# Autodesk Inventor assembly: cabeça_superior
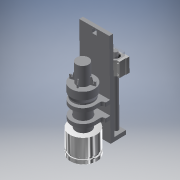
[picture p0: Inventor's stored thumbnail of the model, 180x180]
Saved by Autodesk Inventor 2018 (Build 220112000, 112)
## iProperties
Created: 2018-05-10
Part Number: cabeça_superior
Material: Genérico
Document SubType Name: Assembly
Designer: Georgines
Mass: 943.179 g
Surface Area: 3340.88 cm^2
Volume: 704.097 cm^3
Density: 1.33956 g/cm^3
Author: Georgines
## Documents named in this file (9)
- C:\Users\Georgines\Documents\EstacaoBGA\Peças 3D\cabeça_superior.iam
- C:\Users\Georgines\Documents\EstacaoBGA\Peças 3D\bocal_de_aquecimento.ipt
- C:\Users\Georgines\Documents\EstacaoBGA\Peças 3D\soprador_original.ipt
- C:\Users\Georgines\Documents\EstacaoBGA\Peças 3D\base_fixaxao_cabeca_supeior.ipt
- C:\Users\Georgines\Documents\EstacaoBGA\Peças 3D\carcaca_bocal_superior.ipt
- C:\Users\Georgines\Documents\EstacaoBGA\Peças 3D\SuporteGuiasCabeçasAquecimento.ipt
- C:\Users\Georgines\Documents\EstacaoBGA\Peças 3D\GuiaLinear_12x200mm.ipt
- C:\Users\Georgines\Documents\EstacaoBGA\Peças 3D\SCS12UU.iam
- C:\Users\Georgines\Documents\EstacaoBGA\Peças 3D\SuporteAquecedor.ipt
## Components (12 placed, 8 different names)
1. bocal_de_aquecimento:1 — Coincidência:16, Alinhamento:14, Coincidência:22
2. soprador_original:1 — Coincidência:15, Coincidência:16, Alinhamento:14, Coincidência:17
3. SuporteGuiasCabeçasAquecimento:1 — Coincidência:1, Coincidência:2, Alinhamento:13, Coincidência:19, Coincidência:20, Alinhamento:18, Alinhamento:19
4. SuporteGuiasCabeçasAquecimento:2 — Coincidência:3, Coincidência:4, Coincidência:11, Alinhamento:9, Alinhamento:20
5. GuiaLinear_12x200mm:1 — Coincidência:2, Coincidência:4, Coincidência:10, Alinhamento:19
6. GuiaLinear_12x200mm:2 — Coincidência:1, Coincidência:3, Coincidência:21, Alinhamento:18, Alinhamento:20
7. SCS12UU:1 [sub-assembly] — Coincidência:10, Coincidência:20, Alinhamento:16, Alinhamento:17
8. SCS12UU:4 [sub-assembly] — Coincidência:21, Alinhamento:16, Alinhamento:17
9. base_fixaxao_cabeca_supeior:1 — Coincidência:11, Alinhamento:9, Coincidência:12, Alinhamento:10, Coincidência:13, Alinhamento:11, Alinhamento:12, Alinhamento:13, Coincidência:18, Alinhamento:15, Coincidência:22
10. SuporteAquecedor:1 — Coincidência:12, Alinhamento:10, Alinhamento:12, Coincidência:14, Coincidência:15, Coincidência:17
11. SuporteAquecedor:2 — Coincidência:13, Alinhamento:11, Coincidência:14
12. carcaca_bocal_superior:1 — Coincidência:18, Coincidência:19, Alinhamento:15
## Relationships (29: Mate 17, Flush 12)
- Coincidência:1 [Mate]: SuporteGuiasCabeçasAquecimento:1 ↔ GuiaLinear_12x200mm:2
- Coincidência:2 [Mate]: SuporteGuiasCabeçasAquecimento:1 ↔ GuiaLinear_12x200mm:1
- Coincidência:3 [Mate]: SuporteGuiasCabeçasAquecimento:2 ↔ GuiaLinear_12x200mm:2
- Coincidência:4 [Mate]: SuporteGuiasCabeçasAquecimento:2 ↔ GuiaLinear_12x200mm:1
- Coincidência:10 [Mate]: GuiaLinear_12x200mm:1 ↔ SCS12UU:1
- Coincidência:11 [Mate]: SuporteGuiasCabeçasAquecimento:2 ↔ base_fixaxao_cabeca_supeior:1
- Alinhamento:9 [Flush]: SuporteGuiasCabeçasAquecimento:2 ↔ base_fixaxao_cabeca_supeior:1
- Coincidência:12 [Mate]: base_fixaxao_cabeca_supeior:1 ↔ SuporteAquecedor:1
- Alinhamento:10 [Flush]: base_fixaxao_cabeca_supeior:1 ↔ SuporteAquecedor:1
- Coincidência:13 [Mate]: base_fixaxao_cabeca_supeior:1 ↔ SuporteAquecedor:2
- Alinhamento:11 [Flush]: base_fixaxao_cabeca_supeior:1 ↔ SuporteAquecedor:2
- Alinhamento:12 [Flush] (142.072 mm): base_fixaxao_cabeca_supeior:1 ↔ SuporteAquecedor:1
- Coincidência:14 [Mate] (25.75 mm): SuporteAquecedor:1 ↔ SuporteAquecedor:2
- Alinhamento:13 [Flush]: SuporteGuiasCabeçasAquecimento:1 ↔ base_fixaxao_cabeca_supeior:1
- Coincidência:15 [Mate]: soprador_original:1 ↔ SuporteAquecedor:1
- Coincidência:16 [Mate]: bocal_de_aquecimento:1 ↔ soprador_original:1
- Alinhamento:14 [Flush] (2.5 mm): bocal_de_aquecimento:1 ↔ soprador_original:1
- Coincidência:17 [Mate] (5 mm): soprador_original:1 ↔ SuporteAquecedor:1
- Coincidência:18 [Mate]: base_fixaxao_cabeca_supeior:1 ↔ carcaca_bocal_superior:1
- Coincidência:19 [Mate]: SuporteGuiasCabeçasAquecimento:1 ↔ carcaca_bocal_superior:1
- Alinhamento:15 [Flush]: base_fixaxao_cabeca_supeior:1 ↔ carcaca_bocal_superior:1
- Coincidência:20 [Mate]: SuporteGuiasCabeçasAquecimento:1 ↔ SCS12UU:1
- Coincidência:21 [Mate]: GuiaLinear_12x200mm:2 ↔ SCS12UU:4
- Alinhamento:16 [Flush]: SCS12UU:1 ↔ SCS12UU:4
- Alinhamento:17 [Flush]: SCS12UU:1 ↔ SCS12UU:4
- Coincidência:22 [Mate]: bocal_de_aquecimento:1 ↔ base_fixaxao_cabeca_supeior:1
- Alinhamento:18 [Flush]: SuporteGuiasCabeçasAquecimento:1 ↔ GuiaLinear_12x200mm:2
- Alinhamento:19 [Flush]: SuporteGuiasCabeçasAquecimento:1 ↔ GuiaLinear_12x200mm:1
- Alinhamento:20 [Flush]: SuporteGuiasCabeçasAquecimento:2 ↔ GuiaLinear_12x200mm:2
